# Autodesk Inventor assembly: Test01
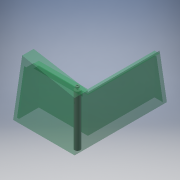
[picture p0: Inventor's stored thumbnail of the model, 180x180]
Saved by Autodesk Inventor 2019 (Build 230136000, 136)
## iProperties
Created: 2019-01-04
Part Number: Test01
Document SubType Name: Assembly
Designer: james
Author: james
## Documents named in this file (5)
- F:\JimsDesign\4089DriversStation\Test01.iam
- F:\JimsDesign\4089DriversStation\FCDLeft1.ipt
- F:\JimsDesign\4089DriversStation\NutDriverShaft.ipt
- F:\JimsDesign\Library\Fasteners\Size-10-32\HexCap-1.ipt
- F:\JimsDesign\Library\Fasteners\Size-10-32\LockNut.ipt
## Components (4 placed, 4 different names)
1. FCDLeft1:1 — Mate:1, Mate:2
2. NutDriverShaft:1 — Mate:1, Mate:4
3. HexCap-1:1 — Mate:2, Mate:3, Mate:4
4. LockNut:1 — Mate:3
## Relationships (4: Mate 4)
- Mate:1: FCDLeft1:1 ↔ NutDriverShaft:1
- Mate:2: FCDLeft1:1 ↔ HexCap-1:1
- Mate:3: HexCap-1:1 ↔ LockNut:1
- Mate:4: NutDriverShaft:1 ↔ HexCap-1:1
